# Autodesk Inventor assembly: Layer2_Ass
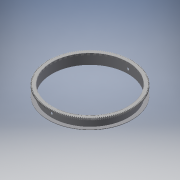
[picture p0: Inventor's stored thumbnail of the model, 180x180]
Saved by Autodesk Inventor 2017 (Build 210142000, 142)
## iProperties
Created: 2017-01-26
Part Number: Layer2_Ass
Document SubType Name: Assembly
Designer: David Kopala
Author: David Kopala
## Documents named in this file (3)
- Z:\Documents\Drone\Drone\3D Models\Project\Chassis_04\Layer2_Ass.iam
- Z:\Documents\Drone\Drone\3D Models\Project\Chassis_04\Layer2.ipt
- Z:\Documents\Drone\Drone\3D Models\Project\Chassis_04\SpurGear_Ref\Design Accelerator\Spur Gear11.ipt
## Components (2 placed, 2 different names)
1. Layer2:1 — Insert:1
2. Spur Gear1:1 — Insert:1
## Relationships (1: Insert 1)
- Insert:1: Layer2:1 ↔ Spur Gear1:1
